# Autodesk Inventor assembly: Băng chuyền
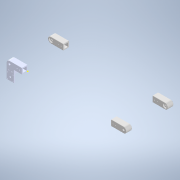
[picture p0: Inventor's stored thumbnail of the model, 180x180]
Saved by Autodesk Inventor 2020 (Build 240168000, 168)
## iProperties
Created: 2022-11-30
Part Number: Băng chuyền
Document SubType Name: Assembly
Designer: ADMIN
Author: ADMIN
## Documents named in this file (3)
- D:\Do-an-tot-nghiep\Inventor\Băng chuyền.iam
- D:\Do-an-tot-nghiep\Inventor\băng chuyền.ipt
- D:\Do-an-tot-nghiep\Inventor\bangchuyenstep.ipt
## Components (4 placed, 2 different names)
1. băng chuyền:1 — Flush:2, Mate:1, Flush:3, Mate:5, Flush:4
2. bangchuyenstep:1 — Flush:1, Flush:3, Mate:4, Mate:5
3. băng chuyền:2 — Flush:2, Mate:1, Mate:2, Mate:3, Flush:4
4. băng chuyền:3 — Flush:1, Mate:2, Mate:3, Mate:4
## Relationships (9: Mate 5, Flush 4)
- Flush:1: bangchuyenstep:1 ↔ băng chuyền:3
- Flush:2: băng chuyền:1 ↔ băng chuyền:2
- Mate:1 (500 mm): băng chuyền:1 ↔ băng chuyền:2
- Flush:3: băng chuyền:1 ↔ bangchuyenstep:1
- Mate:2: băng chuyền:2 ↔ băng chuyền:3
- Mate:3 (200 mm): băng chuyền:2 ↔ băng chuyền:3
- Mate:4 (500 mm): bangchuyenstep:1 ↔ băng chuyền:3
- Mate:5 (200 mm): băng chuyền:1 ↔ bangchuyenstep:1
- Flush:4: băng chuyền:1 ↔ băng chuyền:2
